# Autodesk Inventor assembly: MainTurretAssembly
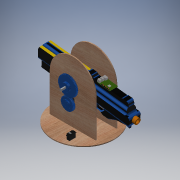
[picture p0: Inventor's stored thumbnail of the model, 180x180]
Saved by Autodesk Inventor 2018 (Build 220112000, 112)
## iProperties
Created: 2019-02-20
Part Number: MainTurretAssembly
Document SubType Name: Assembly
Designer: snipe
Author: snipe
## Documents named in this file (11)
- C:\Users\snipe\Documents\CPRE186-CAD\MainTurretAssembly.iam
- C:\Users\snipe\Documents\CPRE186-CAD\NerfRivalZeus.ipt
- C:\Users\snipe\Documents\CPRE186-CAD\Raspi3B+_Mockup.ipt
- C:\Users\snipe\Documents\CPRE186-CAD\Servo.iam
- C:\Users\snipe\Documents\CPRE186-CAD\turretBasePlate.ipt
- C:\Users\snipe\Documents\CPRE186-CAD\turretSidePlateOne.ipt
- C:\Users\snipe\Documents\CPRE186-CAD\turretSidePlateTwo.ipt
- C:\Users\snipe\Documents\CPRE186-CAD\0.5inHexBearing.ipt
- C:\Users\snipe\Documents\CPRE186-CAD\HexShaft12in.ipt
- C:\Users\snipe\Documents\CPRE186-CAD\gear1.ipt
- C:\Users\snipe\Documents\CPRE186-CAD\gear2.ipt
## Components (12 placed, 10 different names)
1. NerfRivalZeus:1 — Flush:1, Flush:2, Flush:3, Mate:22
2. Raspi3B+_Mockup:1 — Mate:22
3. Servo:1 [sub-assembly] — Mate:16, Mate:17, Mate:18, Mate:19, Mate:20
4. Servo:2 [sub-assembly] — Mate:23
5. turretBasePlate:1 — Mate:1, Mate:2, Mate:3, Mate:4, Mate:5, Mate:6, Mate:23
6. turretSidePlateOne:1 — Mate:1, Mate:2, Mate:3, Mate:7, Mate:8, Symmetry:1, Mate:16, Mate:17, Mate:18
7. turretSidePlateTwo:1 — Mate:4, Mate:5, Mate:6, Mate:9, Mate:10, Symmetry:1
8. 0.5inHexBearing:1 — Mate:7, Mate:8, Mate:11, Mate:12
9. 0.5inHexBearing:2 — Mate:9, Mate:10, Mate:13
10. HexShaft12in:1 — Mate:11, Mate:12, Mate:13, Flush:1, Flush:2, Flush:3, Mate:14, Mate:15
11. gear1:1 — Mate:19, Mate:20, Mate:21, Rotation:1
12. gear2:1 — Mate:14, Mate:15, Mate:21, Rotation:1
## Relationships (28: Mate 23, Flush 3, Symmetry 1, RelateRotation 1)
- Mate:1: turretBasePlate:1 ↔ turretSidePlateOne:1
- Mate:2: turretBasePlate:1 ↔ turretSidePlateOne:1
- Mate:3: turretBasePlate:1 ↔ turretSidePlateOne:1
- Mate:4: turretBasePlate:1 ↔ turretSidePlateTwo:1
- Mate:5: turretBasePlate:1 ↔ turretSidePlateTwo:1
- Mate:6: turretBasePlate:1 ↔ turretSidePlateTwo:1
- Mate:7: turretSidePlateOne:1 ↔ 0.5inHexBearing:1
- Mate:8: turretSidePlateOne:1 ↔ 0.5inHexBearing:1
- Mate:9: turretSidePlateTwo:1 ↔ 0.5inHexBearing:2
- Mate:10: turretSidePlateTwo:1 ↔ 0.5inHexBearing:2
- Mate:11: 0.5inHexBearing:1 ↔ HexShaft12in:1
- Mate:12: 0.5inHexBearing:1 ↔ HexShaft12in:1
- Mate:13: 0.5inHexBearing:2 ↔ HexShaft12in:1
- Flush:1: NerfRivalZeus:1 ↔ HexShaft12in:1
- Flush:2: NerfRivalZeus:1 ↔ HexShaft12in:1
- Flush:3: NerfRivalZeus:1 ↔ HexShaft12in:1
- Symmetry:1: turretSidePlateOne:1 ↔ turretSidePlateTwo:1
- Mate:14: HexShaft12in:1 ↔ gear2:1
- Mate:15: HexShaft12in:1 ↔ gear2:1
- Mate:16: Servo:1 ↔ turretSidePlateOne:1
- Mate:17: Servo:1 ↔ turretSidePlateOne:1
- Mate:18: Servo:1 ↔ turretSidePlateOne:1
- Mate:19: Servo:1 ↔ gear1:1
- Mate:20: Servo:1 ↔ gear1:1
- Mate:21: gear1:1 ↔ gear2:1
- Rotation:1 [RelateRotation] (1 ul): gear1:1 ↔ gear2:1
- Mate:22: NerfRivalZeus:1 ↔ Raspi3B+_Mockup:1
- Mate:23: Servo:2 ↔ turretBasePlate:1
